# Autodesk Inventor assembly: VersaPlanetary v2 Dual Stage 10_1 with RS 550 (1)
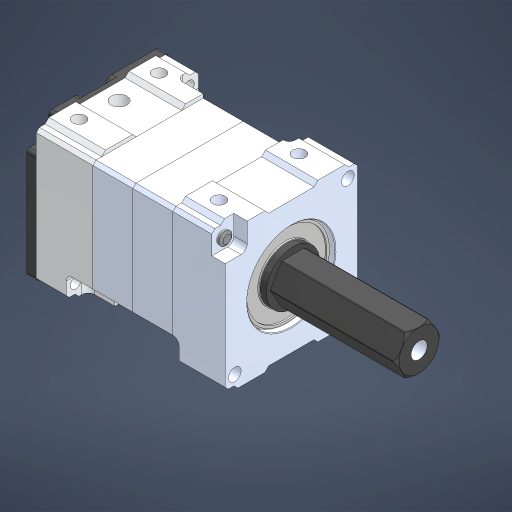
[picture p0: Inventor's stored thumbnail of the model, 512x512]
Saved by Autodesk Inventor 2024.3 (Build 283343000, 343)
## iProperties
Created: 2025-03-17
Part Number: VersaPlanetary v2 Dual Stage 10_1 with RS 550 (1)
Description: STEP AP214
Document SubType Name: Assembly
Designer: Marcus Tannini
Mass: 326.484 g
Surface Area: 544.699 cm^2
Volume: 79.3802 cm^3
Density: 4.11291 g/cm^3
Mfg Approved By: John.Thibert
ILogicPurgeVersion: 0.0.0.0
OnSaveVersion: 3.5.0.0
OnSaveAssembly: COREAutomationManager
Sending System: SolidWorks 2016
Preprocessor: SwSTEP 2.0
ModelCat: Uncategorized
CN_MASS: 0.33
Title: 217-4973_1stage_550.STEP
Revision Number: ANY
## Documents named in this file (15)
- \\clfs\homes\john.thibert\2025-Poseidon-Mechanical\VersaPlanetary v2 Dual Stage 10_1 with RS 550 (1).iam
- \\clfs\homes\john.thibert\2025-Poseidon-Mechanical\217-2625-026 Rev1.ipt
- \\clfs\homes\john.thibert\2025-Poseidon-Mechanical\217-2742-001 Rev4.ipt
- \\clfs\homes\john.thibert\2025-Poseidon-Mechanical\217-2625-017 Rev1_9714K61.ipt
- \\clfs\homes\john.thibert\2025-Poseidon-Mechanical\217-2625-003 Rev1.ipt
- \\clfs\homes\john.thibert\2025-Poseidon-Mechanical\217-2625-018 Rev1_98541A410.ipt
- \\clfs\homes\john.thibert\2025-Poseidon-Mechanical\832-1750-Ring-Gear-Screw_SSA0832-0500ZC.ipt
- \\clfs\homes\john.thibert\2025-Poseidon-Mechanical\217-2625-025 Rev1.ipt
- \\clfs\homes\john.thibert\2025-Poseidon-Mechanical\217-4649-005 Rev1_SSA0003-008BA.ipt
- \\clfs\homes\john.thibert\2025-Poseidon-Mechanical\217-2822-001 Rev4.ipt
- \\clfs\homes\john.thibert\2025-Poseidon-Mechanical\217-2820 Rev1_Public.iam
- \\clfs\homes\john.thibert\2025-Poseidon-Mechanical\217-2816-001 Rev1.ipt
- \\clfs\homes\john.thibert\2025-Poseidon-Mechanical\217-4649-001 Rev1.ipt
- \\clfs\homes\john.thibert\2025-Poseidon-Mechanical\217-4649-007 Rev1_94105A824.ipt
- \\clfs\homes\john.thibert\2025-Poseidon-Mechanical\217-2625-012 Rev1.ipt
## Components (18 placed, 18 different names)
1. 217-2625-026 Rev1_1 — Insert:1, Flush:3
2. 217-2742-001 Rev4_2
3. 217-2742-001 Rev4_3
4. 217-2625-017 Rev1_9714K61_4
5. 217-2625-003 Rev1_5
6. 217-2625-018 Rev1_98541A410_6
7. 832-1750-Ring-Gear-Screw_SSA0832-0500ZC_7
8. 832-1750-Ring-Gear-Screw_SSA0832-0500ZC_8
9. 217-2625-025 Rev1_9 — Insert:3, Flush:1, Mate:1, Mate:2, Flush:4
10. 217-4649-005 Rev1_SSA0003-008BA_12
11. 217-4649-005 Rev1_SSA0003-008BA_13
12. 217-2822-001 Rev4_14 — Mate:1, Mate:2, Flush:4
13. 217-2820 Rev1_Public_16 [sub-assembly]
14. 217-2816-001 Rev1_17 — Insert:2, Insert:3, Flush:1, Flush:2
15. 217-4649-001 Rev1_18
16. 217-4649-007 Rev1_94105A824_19
17. 217-2625-012 Rev1_20
18. 217-2816-001 Rev1:2 — Insert:1, Insert:2, Flush:2, Flush:3
## Relationships (9: Flush 4, Insert 3, Mate 2)
- Insert:1: 217-2625-026 Rev1_1 ↔ 217-2816-001 Rev1:2
- Insert:2: 217-2816-001 Rev1_17 ↔ 217-2816-001 Rev1:2
- Insert:3: 217-2625-025 Rev1_9 ↔ 217-2816-001 Rev1_17
- Flush:1: 217-2625-025 Rev1_9 ↔ 217-2816-001 Rev1_17
- Flush:2: 217-2816-001 Rev1_17 ↔ 217-2816-001 Rev1:2
- Flush:3: 217-2625-026 Rev1_1 ↔ 217-2816-001 Rev1:2
- Mate:1: 217-2625-025 Rev1_9 ↔ 217-2822-001 Rev4_14
- Mate:2: 217-2625-025 Rev1_9 ↔ 217-2822-001 Rev4_14
- Flush:4: 217-2625-025 Rev1_9 ↔ 217-2822-001 Rev4_14
